# Autodesk Inventor assembly: Moving Carousel Assembky
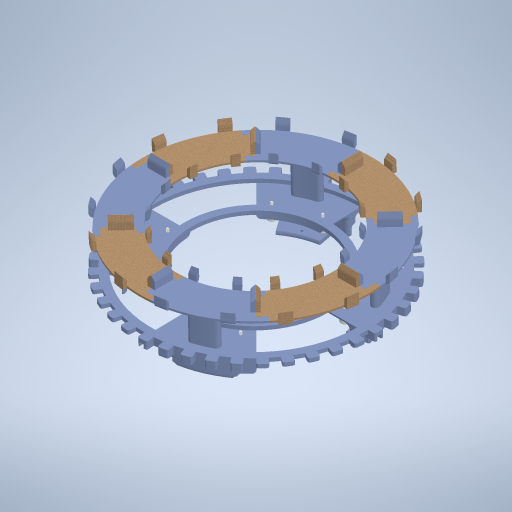
[picture p0: Inventor's stored thumbnail of the model, 512x512]
Saved by Autodesk Inventor 2023 (Build 270158000, 158)
## iProperties
Created: 2023-01-27
Part Number: Moving Carousel Assembky
Document SubType Name: Assembly
Designer: cheng
Author: cheng
## Documents named in this file (3)
- C:\Users\cheng\Desktop\4th Year Project\Inventor\Ninth Assembly\Moving Carousel Assembky.iam
- C:\Users\cheng\Desktop\4th Year Project\Inventor\Ninth Assembly\Moving Carousel Single.iam
- C:\Users\cheng\Desktop\4th Year Project\Inventor\Ninth Assembly\MC_Plate.ipt
## Components (8 placed, 2 different names)
1. Moving Carousel Single:1 [sub-assembly] — Mate:1, Mate:2, Mate:3, Mate:4, Mate:5, Mate:6, Mate:10, Mate:11, Flush:1
2. Moving Carousel Single:2 [sub-assembly] — Mate:7, Mate:8, Mate:9, Mate:12, Mate:15
3. Moving Carousel Single:3 [sub-assembly] — Mate:4, Mate:5, Mate:6, Mate:7, Mate:8, Mate:9, Mate:13, Mate:14
4. Moving Carousel Single:4 [sub-assembly] — Mate:1, Mate:2, Mate:3, Mate:16, Mate:17, Mate:18, Mate:19, Mate:20
5. MC_Plate:1 — Mate:10, Mate:11, Flush:1
6. MC_Plate:2 — Mate:18, Mate:19, Mate:20
7. MC_Plate:3 — Mate:12, Mate:13, Mate:14
8. MC_Plate:4 — Mate:15, Mate:16, Mate:17
## Relationships (21: Mate 20, Flush 1)
- Mate:1: Moving Carousel Single:1 ↔ Moving Carousel Single:4
- Mate:2: Moving Carousel Single:1 ↔ Moving Carousel Single:4
- Mate:3: Moving Carousel Single:1 ↔ Moving Carousel Single:4
- Mate:4: Moving Carousel Single:1 ↔ Moving Carousel Single:3
- Mate:5: Moving Carousel Single:1 ↔ Moving Carousel Single:3
- Mate:6: Moving Carousel Single:1 ↔ Moving Carousel Single:3
- Mate:7: Moving Carousel Single:2 ↔ Moving Carousel Single:3
- Mate:8: Moving Carousel Single:2 ↔ Moving Carousel Single:3
- Mate:9: Moving Carousel Single:2 ↔ Moving Carousel Single:3
- Mate:10: Moving Carousel Single:1 ↔ MC_Plate:1
- Mate:11: Moving Carousel Single:1 ↔ MC_Plate:1
- Flush:1: Moving Carousel Single:1 ↔ MC_Plate:1
- Mate:12: Moving Carousel Single:2 ↔ MC_Plate:3
- Mate:13: Moving Carousel Single:3 ↔ MC_Plate:3
- Mate:14: Moving Carousel Single:3 ↔ MC_Plate:3
- Mate:15: Moving Carousel Single:2 ↔ MC_Plate:4
- Mate:16: Moving Carousel Single:4 ↔ MC_Plate:4
- Mate:17: Moving Carousel Single:4 ↔ MC_Plate:4
- Mate:18: Moving Carousel Single:4 ↔ MC_Plate:2
- Mate:19: Moving Carousel Single:4 ↔ MC_Plate:2
- Mate:20: Moving Carousel Single:4 ↔ MC_Plate:2
